# Autodesk Inventor assembly: base
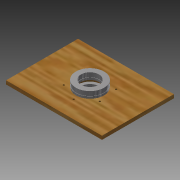
[picture p0: Inventor's stored thumbnail of the model, 180x180]
Saved by Autodesk Inventor 2013 (Build 170138000, 138)
## iProperties
Created: 2014-10-12
Part Number: base
Document SubType Name: Assembly
Designer: Masta
Author: Masta
## Documents named in this file (4)
- D:\DrOctopus\3D model\base.iam
- D:\DrOctopus\3D model\base_plate.ipt
- D:\DrOctopus\3D model\Thrust Bearing 51106 - 30x47x11mm.ipt
- D:\DrOctopus\3D model\Bearing 6006 ZZ - 30x55x13mm.ipt
## Components (3 placed, 3 different names)
1. base_plate:1 — Insert:1, Insert:2
2. Thrust Bearing 51106 - 30x47x11mm:1 — Insert:1
3. Bearing 6006 ZZ - 30x55x13mm:1 — Insert:2
## Relationships (2: Insert 2)
- Insert:1: base_plate:1 ↔ Thrust Bearing 51106 - 30x47x11mm:1
- Insert:2: base_plate:1 ↔ Bearing 6006 ZZ - 30x55x13mm:1
